# Autodesk Inventor assembly: Main Assembly
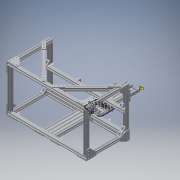
[picture p0: Inventor's stored thumbnail of the model, 180x180]
Saved by Autodesk Inventor 2016 (Build 200138000, 138)
## iProperties
Created: 2016-03-20
Part Number: Main Assembly
Document SubType Name: Assembly
Designer: Solomon
Author: Solomon
## Documents named in this file (13)
- C:\Users\Solomon\Documents\Inventor\SLA MK I\Main Assembly.iam
- C:\Users\Solomon\Documents\Inventor\SLA MK I\V Slot Part Files\Extrusions\vslot 20 x 80 - 500 mm.ipt
- C:\Users\Solomon\Documents\Inventor\SLA MK I\buildplate.iam
- C:\Users\Solomon\Documents\Inventor\SLA MK I\V Slot Part Files\Extrusions\vslot 20 x 20 v2 - 500mm.ipt
- C:\Users\Solomon\Documents\Inventor\SLA MK I\V Slot Part Files\Extrusions\vslot 20 x 20 v2 - 250mm.ipt
- C:\Users\Solomon\Documents\Inventor\SLA MK I\V Slot Part Files\Brackets and Joining Plates\90 Degree Corner Connector.ipt
- C:\Users\Solomon\Documents\Inventor\SLA MK I\V Slot Part Files\Brackets and Joining Plates\5 Hole 90 Degree Bracket.ipt
- C:\Users\Solomon\Documents\Inventor\SLA MK I\V Slot Part Files\Brackets and Joining Plates\3 Hole Joining Strip Plate.ipt
- C:\Users\Solomon\Documents\Inventor\SLA MK I\V Slot Part Files\Brackets and Joining Plates\5 Hole T Joining Plate.ipt
- C:\Users\Solomon\Documents\Inventor\SLA MK I\100mm m5 threaded.ipt
- C:\Users\Solomon\Documents\Inventor\SLA MK I\vwheel.iam
- C:\Users\Solomon\Documents\Inventor\SLA MK I\Motor pulley holder.ipt
- C:\Users\Solomon\Documents\Inventor\SLA MK I\V Slot Part Files\Brackets and Joining Plates\Universal L Bracket.ipt
## Components (71 placed, 12 different names)
1. vslot 20 x 80 - 500 mm:1 — Angle:1, Mate:1, Flush:1, Angle:2, Flush:2, Flush:8, Mate:6, Angle:40, Angle:41, Angle:42, Angle:43, Flush:71, Mate:53, Mate:54, Flush:72, Flush:73, Flush:74, Mate:56, Flush:76, Mate:83, Flush:89, Mate:85, Flush:90, Mate:86, Angle:59, Mate:87, Flush:93, Angle:62, Mate:89, Flush:94, Mate:91
2. buildplate:1 [sub-assembly] — Angle:1, Mate:1, Flush:1, Angle:52, Mate:58, Flush:77, Angle:56, Angle:57
3. vslot 20 x 20 v2 - 500mm:1 — Angle:2, Flush:2, Mate:3, Flush:3, Flush:4, Flush:5, Flush:6, Mate:4, Flush:8, Mate:6, Flush:15, Mate:9, Mate:10, Flush:16, Flush:17, Flush:32, Mate:22, Flush:34, Flush:36, Flush:37, Angle:58, Flush:91, Flush:92
4. vslot 20 x 20 v2 - 500mm:4 — Mate:5, Flush:7, Flush:9, Flush:12, Mate:49, Flush:63, Flush:66, Flush:67, Flush:69, Mate:84, Angle:61, Mate:88, Angle:63, Mate:90, Flush:95
5. vslot 20 x 20 v2 - 250mm:1 — Mate:3, Flush:3, Flush:4, Flush:9, Angle:6, Mate:7, Flush:10, Flush:11, Angle:15, Flush:31, Mate:21, Angle:16, Flush:33, Angle:28, Mate:52, Mate:69, Flush:82
6. vslot 20 x 20 v2 - 250mm:2 — Flush:5, Flush:6, Mate:4, Mate:5, Flush:7, Angle:3, Angle:4, Angle:5, Flush:13, Mate:8, Flush:14, Mate:12, Angle:17, Angle:18, Flush:35, Mate:23, Flush:38, Mate:24, Angle:37, Mate:50, Flush:65, Angle:38, Mate:51, Mate:71, Flush:83
7. vslot 20 x 20 v2 - 250mm:3 — Angle:6, Mate:7, Flush:10, Flush:11, Angle:7, Angle:8, Mate:11, Flush:29, Flush:30, Angle:25, Angle:27, Flush:47, Flush:64, Flush:70, Mate:64, Flush:80, Mate:66, Flush:81, Mate:67, Mate:75, Mate:77
8. vslot 20 x 20 v2 - 250mm:4 — Angle:4, Flush:12, Flush:13, Mate:8, Flush:18, Flush:19, Mate:13, Angle:13, Angle:19, Flush:68, Angle:53, Mate:60, Angle:54, Mate:62, Mate:73, Mate:79, Mate:82
9. vslot 20 x 20 v2 - 250mm:5 — Angle:5, Flush:14, Flush:15, Mate:9, Flush:24, Mate:19, Flush:25
10. vslot 20 x 20 v2 - 250mm:6 — Angle:3, Mate:10, Flush:16, Flush:17, Flush:45
11. vslot 20 x 20 v2 - 500mm:5 — Angle:7, Flush:24, Mate:19, Flush:25, Flush:26, Flush:27, Mate:20, Flush:28, Flush:40, Flush:43, Flush:46, Mate:32, Mate:34, Mate:36, Mate:39
12. vslot 20 x 20 v2 - 500mm:6 — Angle:8, Mate:11, Flush:18, Mate:12, Mate:15, Mate:16, Flush:22, Flush:23, Mate:68, Mate:70, Mate:72, Mate:74, Flush:86, Mate:78, Flush:87, Mate:80
13. vslot 20 x 20 v2 - 500mm:7 — Flush:19, Mate:13, Angle:9, Mate:17, Mate:18, Flush:20, Flush:21, Mate:59, Flush:78, Angle:55, Mate:61, Mate:63, Flush:79, Mate:65, Flush:85, Mate:76, Mate:81, Flush:88
14. 90 Degree Corner Connector:1 — Angle:12, Mate:18, Angle:13, Flush:20, Angle:14
15. 90 Degree Corner Connector:2 — Angle:11, Angle:12, Mate:17, Flush:21
16. 90 Degree Corner Connector:3 — Angle:9, Angle:10, Angle:11, Mate:15, Flush:22
17. 90 Degree Corner Connector:4 — Angle:10, Mate:16, Angle:14, Flush:23
18. vslot 20 x 20 v2 - 250mm:7 — Flush:26, Flush:27, Mate:20, Angle:20, Angle:21, Flush:39, Mate:25, Angle:22, Angle:23, Flush:41, Mate:26, Angle:29, Angle:30, Mate:30, Flush:49, Flush:50, Mate:31, Mate:46, Mate:48
19. vslot 20 x 20 v2 - 250mm:8 — Flush:28, Flush:29, Flush:30, Angle:24, Flush:44, Mate:27, Angle:26, Mate:28, Flush:48, Mate:29, Flush:51, Flush:52, Mate:33, Mate:42, Mate:44
20. 5 Hole 90 Degree Bracket:1 — Angle:19, Flush:37, Flush:38, Mate:24
21. 5 Hole 90 Degree Bracket:4 — Angle:17, Angle:18, Flush:35, Flush:36, Mate:23
22. 5 Hole 90 Degree Bracket:5 — Angle:16, Flush:33, Mate:22, Flush:34
23. 5 Hole 90 Degree Bracket:6 — Angle:15, Flush:31, Flush:32, Mate:21
24. 5 Hole 90 Degree Bracket:7 — Angle:20, Angle:21, Flush:39, Flush:40, Mate:25, Flush:42
25. 5 Hole 90 Degree Bracket:8 — Angle:22, Angle:23, Flush:41, Flush:42, Mate:26
26. 5 Hole 90 Degree Bracket:9 — Angle:24, Flush:43, Flush:44, Mate:27
27. 5 Hole 90 Degree Bracket:10 — Angle:25, Angle:26, Mate:28, Flush:45, Flush:46
28. 5 Hole 90 Degree Bracket:11 — Angle:27, Angle:28, Flush:47, Flush:48, Mate:29, Angle:31
29. 5 Hole 90 Degree Bracket:13 — Angle:29, Angle:30, Mate:30, Flush:49, Flush:50
30. 3 Hole Joining Strip Plate 3 Hole Joining Strip Plate:1 — Angle:33, Angle:34, Mate:35, Flush:53, Mate:36, Flush:54, Flush:55
31. vslot 20 x 20 v2 - 250mm:9 — Angle:31, Flush:51, Mate:31, Mate:32, Angle:32, Angle:35, Mate:38, Flush:56, Mate:40, Angle:36, Mate:45, Flush:61, Mate:47, Flush:62
32. vslot 20 x 20 v2 - 250mm:10 — Angle:32, Flush:52, Mate:33, Mate:34, Angle:33, Angle:34, Mate:35, Flush:53, Mate:37, Mate:41, Flush:59, Mate:43, Flush:60
33. 3 Hole Joining Strip Plate 3 Hole Joining Strip Plate:5 — Mate:37, Flush:54, Flush:55
34. 3 Hole Joining Strip Plate 3 Hole Joining Strip Plate:6 — Angle:35, Mate:38, Flush:56, Mate:39, Flush:57, Flush:58
35. 3 Hole Joining Strip Plate 3 Hole Joining Strip Plate:7 — Mate:40, Flush:57, Flush:58
36. 3 Hole Joining Strip Plate 3 Hole Joining Strip Plate:8 — Mate:41, Flush:59, Mate:42
37. 3 Hole Joining Strip Plate 3 Hole Joining Strip Plate:9 — Mate:43, Mate:44, Flush:60
38. 3 Hole Joining Strip Plate 3 Hole Joining Strip Plate:10 — Angle:36, Mate:45, Flush:61, Mate:46
39. 3 Hole Joining Strip Plate 3 Hole Joining Strip Plate:11 — Mate:47, Flush:62, Mate:48
40. 5 Hole 90 Degree Bracket:14 — Mate:49, Flush:63, Flush:64
41. 5 Hole 90 Degree Bracket:15 — Angle:37, Mate:50, Flush:65, Flush:66, Angle:39
42. 5 Hole T Joining Plate:1 — Angle:38, Angle:39, Mate:51, Flush:67, Flush:68
43. 5 Hole T Joining Plate:2 — Mate:52, Flush:69, Flush:70
44. 3 Hole Joining Strip Plate 3 Hole Joining Strip Plate:12 — Angle:40, Angle:41, Mate:54, Flush:72, Flush:73, Mate:57, Flush:75
45. 3 Hole Joining Strip Plate 3 Hole Joining Strip Plate:13 — Angle:42, Angle:43, Flush:71, Mate:53, Flush:74, Angle:44, Mate:55, Insert:1, Angle:49, Angle:50, Angle:51
46. 3 Hole Joining Strip Plate 3 Hole Joining Strip Plate:14 — Angle:44, Angle:45, Mate:55, Flush:76, Angle:46, Angle:47, Angle:48, Insert:2, Insert:3, Mate:85
47. 3 Hole Joining Strip Plate 3 Hole Joining Strip Plate:15 — Angle:45, Mate:56, Mate:57, Flush:75
48. 100mm m5 threaded:1 — Angle:48, Insert:3, Insert:5
49. 100mm m5 threaded:2 — Angle:47, Insert:2, Insert:6
50. 100mm m5 threaded:3 — Angle:46, Insert:1, Insert:4
51. vwheel:1 [sub-assembly] — Angle:50, Insert:5
52. vwheel:2 [sub-assembly] — Angle:49, Insert:6
53. vwheel:3 [sub-assembly] — Angle:51, Insert:4
54. 5 Hole T Joining Plate:3 — Angle:52, Mate:58, Flush:77
55. 90 Degree Corner Connector:5 — Angle:53, Mate:59, Mate:60, Flush:78
56. 90 Degree Corner Connector:6 — Angle:54, Angle:55, Mate:61, Mate:62
57. 90 Degree Corner Connector:7 — Mate:63, Mate:64, Flush:79
58. 90 Degree Corner Connector:8 — Flush:80, Mate:65, Mate:66
59. 90 Degree Corner Connector:9 — Flush:81, Mate:67, Mate:68
60. 90 Degree Corner Connector:10 — Mate:69, Flush:82, Mate:70
61. 90 Degree Corner Connector:11 — Mate:71, Flush:83, Mate:72, Flush:84
62. 90 Degree Corner Connector:12 — Flush:84, Mate:73, Mate:74
63. 90 Degree Corner Connector:13 — Mate:75, Flush:85, Mate:76
64. 90 Degree Corner Connector:14 — Mate:77, Flush:86, Mate:78
65. 90 Degree Corner Connector:15 — Flush:87, Mate:79, Mate:80
66. 90 Degree Corner Connector:16 — Mate:81, Mate:82, Flush:88
67. Motor pulley holder:1 — Angle:56, Mate:83, Angle:57, Flush:89, Mate:84
68. 5 Hole 90 Degree Bracket:16 — Angle:59, Angle:60, Flush:92, Mate:87, Flush:93
69. 5 Hole 90 Degree Bracket:17 — Angle:58, Flush:90, Mate:86, Flush:91, Angle:60
70. Universal L Bracket:1 — Angle:61, Angle:62, Mate:88, Mate:89, Flush:94
71. 90 Degree Corner Connector:17 — Angle:63, Mate:90, Flush:95, Mate:91
## Relationships (253: Flush 95, Mate 89, Angle 63, Insert 6)
- Angle:1 (0 deg): vslot 20 x 80 - 500 mm:1 ↔ buildplate:1
- Mate:1 (1.5 mm): vslot 20 x 80 - 500 mm:1 ↔ buildplate:1
- Flush:1 (-23.5 mm): vslot 20 x 80 - 500 mm:1 ↔ buildplate:1
- Angle:2 (0 deg): vslot 20 x 80 - 500 mm:1 ↔ vslot 20 x 20 v2 - 500mm:1
- Flush:2 (-210 mm): vslot 20 x 80 - 500 mm:1 ↔ vslot 20 x 20 v2 - 500mm:1
- Mate:3: vslot 20 x 20 v2 - 500mm:1 ↔ vslot 20 x 20 v2 - 250mm:1
- Flush:3: vslot 20 x 20 v2 - 500mm:1 ↔ vslot 20 x 20 v2 - 250mm:1
- Flush:4: vslot 20 x 20 v2 - 500mm:1 ↔ vslot 20 x 20 v2 - 250mm:1
- Flush:5: vslot 20 x 20 v2 - 500mm:1 ↔ vslot 20 x 20 v2 - 250mm:2
- Flush:6: vslot 20 x 20 v2 - 500mm:1 ↔ vslot 20 x 20 v2 - 250mm:2
- Mate:4: vslot 20 x 20 v2 - 500mm:1 ↔ vslot 20 x 20 v2 - 250mm:2
- Mate:5: vslot 20 x 20 v2 - 500mm:4 ↔ vslot 20 x 20 v2 - 250mm:2
- Flush:7: vslot 20 x 20 v2 - 500mm:4 ↔ vslot 20 x 20 v2 - 250mm:2
- Flush:8: vslot 20 x 80 - 500 mm:1 ↔ vslot 20 x 20 v2 - 500mm:1
- Mate:6: vslot 20 x 80 - 500 mm:1 ↔ vslot 20 x 20 v2 - 500mm:1
- Flush:9: vslot 20 x 20 v2 - 500mm:4 ↔ vslot 20 x 20 v2 - 250mm:1
- Angle:3 (0 deg): vslot 20 x 20 v2 - 250mm:2 ↔ vslot 20 x 20 v2 - 250mm:6
- Angle:4 (0 deg): vslot 20 x 20 v2 - 250mm:2 ↔ vslot 20 x 20 v2 - 250mm:4
- Angle:5 (0 deg): vslot 20 x 20 v2 - 250mm:2 ↔ vslot 20 x 20 v2 - 250mm:5
- Angle:6 (0 deg): vslot 20 x 20 v2 - 250mm:1 ↔ vslot 20 x 20 v2 - 250mm:3
- Mate:7: vslot 20 x 20 v2 - 250mm:1 ↔ vslot 20 x 20 v2 - 250mm:3
- Flush:10: vslot 20 x 20 v2 - 250mm:1 ↔ vslot 20 x 20 v2 - 250mm:3
- Flush:11: vslot 20 x 20 v2 - 250mm:1 ↔ vslot 20 x 20 v2 - 250mm:3
- Flush:12: vslot 20 x 20 v2 - 500mm:4 ↔ vslot 20 x 20 v2 - 250mm:4
- Flush:13: vslot 20 x 20 v2 - 250mm:2 ↔ vslot 20 x 20 v2 - 250mm:4
- Mate:8: vslot 20 x 20 v2 - 250mm:2 ↔ vslot 20 x 20 v2 - 250mm:4
- Flush:14: vslot 20 x 20 v2 - 250mm:2 ↔ vslot 20 x 20 v2 - 250mm:5
- Flush:15: vslot 20 x 20 v2 - 500mm:1 ↔ vslot 20 x 20 v2 - 250mm:5
- Mate:9: vslot 20 x 20 v2 - 500mm:1 ↔ vslot 20 x 20 v2 - 250mm:5
- Mate:10: vslot 20 x 20 v2 - 500mm:1 ↔ vslot 20 x 20 v2 - 250mm:6
- Flush:16: vslot 20 x 20 v2 - 500mm:1 ↔ vslot 20 x 20 v2 - 250mm:6
- Flush:17: vslot 20 x 20 v2 - 500mm:1 ↔ vslot 20 x 20 v2 - 250mm:6
- Angle:7 (0 deg): vslot 20 x 20 v2 - 250mm:3 ↔ vslot 20 x 20 v2 - 500mm:5
- Angle:8 (0 deg): vslot 20 x 20 v2 - 250mm:3 ↔ vslot 20 x 20 v2 - 500mm:6
- Mate:11: vslot 20 x 20 v2 - 250mm:3 ↔ vslot 20 x 20 v2 - 500mm:6
- Flush:18: vslot 20 x 20 v2 - 250mm:4 ↔ vslot 20 x 20 v2 - 500mm:6
- Mate:12: vslot 20 x 20 v2 - 250mm:2 ↔ vslot 20 x 20 v2 - 500mm:6
- Flush:19: vslot 20 x 20 v2 - 250mm:4 ↔ vslot 20 x 20 v2 - 500mm:7
- Mate:13: vslot 20 x 20 v2 - 250mm:4 ↔ vslot 20 x 20 v2 - 500mm:7
- Angle:9 (180 deg): vslot 20 x 20 v2 - 500mm:7 ↔ 90 Degree Corner Connector:3
- Angle:10 (0 deg): 90 Degree Corner Connector:3 ↔ 90 Degree Corner Connector:4
- Angle:11 (0 deg): 90 Degree Corner Connector:2 ↔ 90 Degree Corner Connector:3
- Angle:12 (0 deg): 90 Degree Corner Connector:1 ↔ 90 Degree Corner Connector:2
- Mate:15: vslot 20 x 20 v2 - 500mm:6 ↔ 90 Degree Corner Connector:3
- Mate:16: vslot 20 x 20 v2 - 500mm:6 ↔ 90 Degree Corner Connector:4
- Mate:17: vslot 20 x 20 v2 - 500mm:7 ↔ 90 Degree Corner Connector:2
- Mate:18: vslot 20 x 20 v2 - 500mm:7 ↔ 90 Degree Corner Connector:1
- Angle:13 (0 deg): vslot 20 x 20 v2 - 250mm:4 ↔ 90 Degree Corner Connector:1
- Flush:20: vslot 20 x 20 v2 - 500mm:7 ↔ 90 Degree Corner Connector:1
- Flush:21: vslot 20 x 20 v2 - 500mm:7 ↔ 90 Degree Corner Connector:2
- Flush:22: vslot 20 x 20 v2 - 500mm:6 ↔ 90 Degree Corner Connector:3
- Angle:14 (0 deg): 90 Degree Corner Connector:1 ↔ 90 Degree Corner Connector:4
- Flush:23: vslot 20 x 20 v2 - 500mm:6 ↔ 90 Degree Corner Connector:4
- Flush:24: vslot 20 x 20 v2 - 250mm:5 ↔ vslot 20 x 20 v2 - 500mm:5
- Mate:19: vslot 20 x 20 v2 - 250mm:5 ↔ vslot 20 x 20 v2 - 500mm:5
- Flush:25: vslot 20 x 20 v2 - 250mm:5 ↔ vslot 20 x 20 v2 - 500mm:5
- Flush:26: vslot 20 x 20 v2 - 500mm:5 ↔ vslot 20 x 20 v2 - 250mm:7
- Flush:27: vslot 20 x 20 v2 - 500mm:5 ↔ vslot 20 x 20 v2 - 250mm:7
- Mate:20: vslot 20 x 20 v2 - 500mm:5 ↔ vslot 20 x 20 v2 - 250mm:7
- Flush:28: vslot 20 x 20 v2 - 500mm:5 ↔ vslot 20 x 20 v2 - 250mm:8
- Flush:29: vslot 20 x 20 v2 - 250mm:3 ↔ vslot 20 x 20 v2 - 250mm:8
- Flush:30: vslot 20 x 20 v2 - 250mm:3 ↔ vslot 20 x 20 v2 - 250mm:8
- Angle:15 (0 deg): vslot 20 x 20 v2 - 250mm:1 ↔ 5 Hole 90 Degree Bracket:6
- Flush:31: vslot 20 x 20 v2 - 250mm:1 ↔ 5 Hole 90 Degree Bracket:6
- Flush:32: vslot 20 x 20 v2 - 500mm:1 ↔ 5 Hole 90 Degree Bracket:6
- Mate:21: vslot 20 x 20 v2 - 250mm:1 ↔ 5 Hole 90 Degree Bracket:6
- Angle:16 (0 deg): vslot 20 x 20 v2 - 250mm:1 ↔ 5 Hole 90 Degree Bracket:5
- Flush:33: vslot 20 x 20 v2 - 250mm:1 ↔ 5 Hole 90 Degree Bracket:5
- Mate:22: vslot 20 x 20 v2 - 500mm:1 ↔ 5 Hole 90 Degree Bracket:5
- Flush:34: vslot 20 x 20 v2 - 500mm:1 ↔ 5 Hole 90 Degree Bracket:5
- Angle:17 (0 deg): vslot 20 x 20 v2 - 250mm:2 ↔ 5 Hole 90 Degree Bracket:4
- Angle:18 (0 deg): vslot 20 x 20 v2 - 250mm:2 ↔ 5 Hole 90 Degree Bracket:4
- Flush:35: vslot 20 x 20 v2 - 250mm:2 ↔ 5 Hole 90 Degree Bracket:4
- Flush:36: vslot 20 x 20 v2 - 500mm:1 ↔ 5 Hole 90 Degree Bracket:4
- Mate:23: vslot 20 x 20 v2 - 250mm:2 ↔ 5 Hole 90 Degree Bracket:4
- Angle:19 (0 deg): vslot 20 x 20 v2 - 250mm:4 ↔ 5 Hole 90 Degree Bracket:1
- Flush:37: vslot 20 x 20 v2 - 500mm:1 ↔ 5 Hole 90 Degree Bracket:1
- Flush:38: vslot 20 x 20 v2 - 250mm:2 ↔ 5 Hole 90 Degree Bracket:1
- Mate:24: vslot 20 x 20 v2 - 250mm:2 ↔ 5 Hole 90 Degree Bracket:1
- Angle:20 (0 deg): vslot 20 x 20 v2 - 250mm:7 ↔ 5 Hole 90 Degree Bracket:7
- Angle:21 (0 deg): vslot 20 x 20 v2 - 250mm:7 ↔ 5 Hole 90 Degree Bracket:7
- Flush:39: vslot 20 x 20 v2 - 250mm:7 ↔ 5 Hole 90 Degree Bracket:7
- Flush:40: vslot 20 x 20 v2 - 500mm:5 ↔ 5 Hole 90 Degree Bracket:7
- Mate:25: vslot 20 x 20 v2 - 250mm:7 ↔ 5 Hole 90 Degree Bracket:7
- Angle:22 (0 deg): vslot 20 x 20 v2 - 250mm:7 ↔ 5 Hole 90 Degree Bracket:8
- Angle:23 (0 deg): vslot 20 x 20 v2 - 250mm:7 ↔ 5 Hole 90 Degree Bracket:8
- Flush:41: vslot 20 x 20 v2 - 250mm:7 ↔ 5 Hole 90 Degree Bracket:8
- Flush:42: 5 Hole 90 Degree Bracket:7 ↔ 5 Hole 90 Degree Bracket:8
- Mate:26: vslot 20 x 20 v2 - 250mm:7 ↔ 5 Hole 90 Degree Bracket:8
- Angle:24 (0 deg): vslot 20 x 20 v2 - 250mm:8 ↔ 5 Hole 90 Degree Bracket:9
- Flush:43: vslot 20 x 20 v2 - 500mm:5 ↔ 5 Hole 90 Degree Bracket:9
- Flush:44: vslot 20 x 20 v2 - 250mm:8 ↔ 5 Hole 90 Degree Bracket:9
- Mate:27: vslot 20 x 20 v2 - 250mm:8 ↔ 5 Hole 90 Degree Bracket:9
- Angle:25 (0 deg): vslot 20 x 20 v2 - 250mm:3 ↔ 5 Hole 90 Degree Bracket:10
- Angle:26 (180 deg): vslot 20 x 20 v2 - 250mm:8 ↔ 5 Hole 90 Degree Bracket:10
- Mate:28: vslot 20 x 20 v2 - 250mm:8 ↔ 5 Hole 90 Degree Bracket:10
- Flush:45: vslot 20 x 20 v2 - 250mm:6 ↔ 5 Hole 90 Degree Bracket:10
- Flush:46: vslot 20 x 20 v2 - 500mm:5 ↔ 5 Hole 90 Degree Bracket:10
- Angle:27 (0 deg): vslot 20 x 20 v2 - 250mm:3 ↔ 5 Hole 90 Degree Bracket:11
- Angle:28 (0 deg): vslot 20 x 20 v2 - 250mm:1 ↔ 5 Hole 90 Degree Bracket:11
- Flush:47: vslot 20 x 20 v2 - 250mm:3 ↔ 5 Hole 90 Degree Bracket:11
- Flush:48: vslot 20 x 20 v2 - 250mm:8 ↔ 5 Hole 90 Degree Bracket:11
- Mate:29: vslot 20 x 20 v2 - 250mm:8 ↔ 5 Hole 90 Degree Bracket:11
- Angle:29 (0 deg): vslot 20 x 20 v2 - 250mm:7 ↔ 5 Hole 90 Degree Bracket:13
- Angle:30 (180 deg): vslot 20 x 20 v2 - 250mm:7 ↔ 5 Hole 90 Degree Bracket:13
- Mate:30: vslot 20 x 20 v2 - 250mm:7 ↔ 5 Hole 90 Degree Bracket:13
- Flush:49: vslot 20 x 20 v2 - 250mm:7 ↔ 5 Hole 90 Degree Bracket:13
- Flush:50: vslot 20 x 20 v2 - 250mm:7 ↔ 5 Hole 90 Degree Bracket:13
- Angle:31 (45 deg): 5 Hole 90 Degree Bracket:11 ↔ vslot 20 x 20 v2 - 250mm:9
- Flush:51: vslot 20 x 20 v2 - 250mm:8 ↔ vslot 20 x 20 v2 - 250mm:9
- Mate:31: vslot 20 x 20 v2 - 250mm:7 ↔ vslot 20 x 20 v2 - 250mm:9
- Mate:32: vslot 20 x 20 v2 - 500mm:5 ↔ vslot 20 x 20 v2 - 250mm:9
- Angle:32 (90 deg): vslot 20 x 20 v2 - 250mm:9 ↔ vslot 20 x 20 v2 - 250mm:10
- Flush:52: vslot 20 x 20 v2 - 250mm:8 ↔ vslot 20 x 20 v2 - 250mm:10
- Mate:33: vslot 20 x 20 v2 - 250mm:8 ↔ vslot 20 x 20 v2 - 250mm:10
- Mate:34: vslot 20 x 20 v2 - 500mm:5 ↔ vslot 20 x 20 v2 - 250mm:10
- Angle:33 (0 deg): 3 Hole Joining Strip Plate 3 Hole Joining Strip Plate:1 ↔ vslot 20 x 20 v2 - 250mm:10
- Angle:34 (0 deg): 3 Hole Joining Strip Plate 3 Hole Joining Strip Plate:1 ↔ vslot 20 x 20 v2 - 250mm:10
- Mate:35: 3 Hole Joining Strip Plate 3 Hole Joining Strip Plate:1 ↔ vslot 20 x 20 v2 - 250mm:10
- Flush:53: 3 Hole Joining Strip Plate 3 Hole Joining Strip Plate:1 ↔ vslot 20 x 20 v2 - 250mm:10
- Mate:36: vslot 20 x 20 v2 - 500mm:5 ↔ 3 Hole Joining Strip Plate 3 Hole Joining Strip Plate:1
- Mate:37: vslot 20 x 20 v2 - 250mm:10 ↔ 3 Hole Joining Strip Plate 3 Hole Joining Strip Plate:5
- Flush:54: 3 Hole Joining Strip Plate 3 Hole Joining Strip Plate:1 ↔ 3 Hole Joining Strip Plate 3 Hole Joining Strip Plate:5
- Flush:55: 3 Hole Joining Strip Plate 3 Hole Joining Strip Plate:1 ↔ 3 Hole Joining Strip Plate 3 Hole Joining Strip Plate:5
- Angle:35 (0 deg): vslot 20 x 20 v2 - 250mm:9 ↔ 3 Hole Joining Strip Plate 3 Hole Joining Strip Plate:6
- Mate:38: vslot 20 x 20 v2 - 250mm:9 ↔ 3 Hole Joining Strip Plate 3 Hole Joining Strip Plate:6
- Flush:56: vslot 20 x 20 v2 - 250mm:9 ↔ 3 Hole Joining Strip Plate 3 Hole Joining Strip Plate:6
- Mate:39: vslot 20 x 20 v2 - 500mm:5 ↔ 3 Hole Joining Strip Plate 3 Hole Joining Strip Plate:6
- Mate:40: vslot 20 x 20 v2 - 250mm:9 ↔ 3 Hole Joining Strip Plate 3 Hole Joining Strip Plate:7
- Flush:57: 3 Hole Joining Strip Plate 3 Hole Joining Strip Plate:6 ↔ 3 Hole Joining Strip Plate 3 Hole Joining Strip Plate:7
- Flush:58: 3 Hole Joining Strip Plate 3 Hole Joining Strip Plate:6 ↔ 3 Hole Joining Strip Plate 3 Hole Joining Strip Plate:7
- Mate:41: vslot 20 x 20 v2 - 250mm:10 ↔ 3 Hole Joining Strip Plate 3 Hole Joining Strip Plate:8
- Flush:59: vslot 20 x 20 v2 - 250mm:10 ↔ 3 Hole Joining Strip Plate 3 Hole Joining Strip Plate:8
- Mate:42: vslot 20 x 20 v2 - 250mm:8 ↔ 3 Hole Joining Strip Plate 3 Hole Joining Strip Plate:8
- Mate:43: vslot 20 x 20 v2 - 250mm:10 ↔ 3 Hole Joining Strip Plate 3 Hole Joining Strip Plate:9
- Mate:44: vslot 20 x 20 v2 - 250mm:8 ↔ 3 Hole Joining Strip Plate 3 Hole Joining Strip Plate:9
- Flush:60: vslot 20 x 20 v2 - 250mm:10 ↔ 3 Hole Joining Strip Plate 3 Hole Joining Strip Plate:9
- Angle:36 (0 deg): vslot 20 x 20 v2 - 250mm:9 ↔ 3 Hole Joining Strip Plate 3 Hole Joining Strip Plate:10
- Mate:45: vslot 20 x 20 v2 - 250mm:9 ↔ 3 Hole Joining Strip Plate 3 Hole Joining Strip Plate:10
- Flush:61: vslot 20 x 20 v2 - 250mm:9 ↔ 3 Hole Joining Strip Plate 3 Hole Joining Strip Plate:10
- Mate:46: vslot 20 x 20 v2 - 250mm:7 ↔ 3 Hole Joining Strip Plate 3 Hole Joining Strip Plate:10
- Mate:47: vslot 20 x 20 v2 - 250mm:9 ↔ 3 Hole Joining Strip Plate 3 Hole Joining Strip Plate:11
- Flush:62: vslot 20 x 20 v2 - 250mm:9 ↔ 3 Hole Joining Strip Plate 3 Hole Joining Strip Plate:11
- Mate:48: vslot 20 x 20 v2 - 250mm:7 ↔ 3 Hole Joining Strip Plate 3 Hole Joining Strip Plate:11
- Mate:49: vslot 20 x 20 v2 - 500mm:4 ↔ 5 Hole 90 Degree Bracket:14
- Flush:63: vslot 20 x 20 v2 - 500mm:4 ↔ 5 Hole 90 Degree Bracket:14
- Flush:64: vslot 20 x 20 v2 - 250mm:3 ↔ 5 Hole 90 Degree Bracket:14
- Angle:37 (0 deg): vslot 20 x 20 v2 - 250mm:2 ↔ 5 Hole 90 Degree Bracket:15
- Mate:50: vslot 20 x 20 v2 - 250mm:2 ↔ 5 Hole 90 Degree Bracket:15
- Flush:65: vslot 20 x 20 v2 - 250mm:2 ↔ 5 Hole 90 Degree Bracket:15
- Flush:66: vslot 20 x 20 v2 - 500mm:4 ↔ 5 Hole 90 Degree Bracket:15
- Angle:38 (0 deg): vslot 20 x 20 v2 - 250mm:2 ↔ 5 Hole T Joining Plate:1
- Angle:39 (0 deg): 5 Hole 90 Degree Bracket:15 ↔ 5 Hole T Joining Plate:1
- Mate:51: vslot 20 x 20 v2 - 250mm:2 ↔ 5 Hole T Joining Plate:1
- Flush:67: vslot 20 x 20 v2 - 500mm:4 ↔ 5 Hole T Joining Plate:1
- Flush:68: vslot 20 x 20 v2 - 250mm:4 ↔ 5 Hole T Joining Plate:1
- Mate:52: vslot 20 x 20 v2 - 250mm:1 ↔ 5 Hole T Joining Plate:2
- Flush:69: vslot 20 x 20 v2 - 500mm:4 ↔ 5 Hole T Joining Plate:2
- Flush:70: vslot 20 x 20 v2 - 250mm:3 ↔ 5 Hole T Joining Plate:2
- Angle:40 (0 deg): vslot 20 x 80 - 500 mm:1 ↔ 3 Hole Joining Strip Plate 3 Hole Joining Strip Plate:12
- Angle:41 (0 deg): vslot 20 x 80 - 500 mm:1 ↔ 3 Hole Joining Strip Plate 3 Hole Joining Strip Plate:12
- Angle:42 (0 deg): vslot 20 x 80 - 500 mm:1 ↔ 3 Hole Joining Strip Plate 3 Hole Joining Strip Plate:13
- Angle:43 (0 deg): vslot 20 x 80 - 500 mm:1 ↔ 3 Hole Joining Strip Plate 3 Hole Joining Strip Plate:13
- Flush:71: vslot 20 x 80 - 500 mm:1 ↔ 3 Hole Joining Strip Plate 3 Hole Joining Strip Plate:13
- Mate:53: vslot 20 x 80 - 500 mm:1 ↔ 3 Hole Joining Strip Plate 3 Hole Joining Strip Plate:13
- Mate:54: vslot 20 x 80 - 500 mm:1 ↔ 3 Hole Joining Strip Plate 3 Hole Joining Strip Plate:12
- Flush:72: vslot 20 x 80 - 500 mm:1 ↔ 3 Hole Joining Strip Plate 3 Hole Joining Strip Plate:12
- Flush:73 (-25 mm): vslot 20 x 80 - 500 mm:1 ↔ 3 Hole Joining Strip Plate 3 Hole Joining Strip Plate:12
- Flush:74 (-25 mm): vslot 20 x 80 - 500 mm:1 ↔ 3 Hole Joining Strip Plate 3 Hole Joining Strip Plate:13
- Angle:44 (0 deg): 3 Hole Joining Strip Plate 3 Hole Joining Strip Plate:13 ↔ 3 Hole Joining Strip Plate 3 Hole Joining Strip Plate:14
- Angle:45 (0 deg): 3 Hole Joining Strip Plate 3 Hole Joining Strip Plate:14 ↔ 3 Hole Joining Strip Plate 3 Hole Joining Strip Plate:15
- Mate:55: 3 Hole Joining Strip Plate 3 Hole Joining Strip Plate:13 ↔ 3 Hole Joining Strip Plate 3 Hole Joining Strip Plate:14
- Mate:56: vslot 20 x 80 - 500 mm:1 ↔ 3 Hole Joining Strip Plate 3 Hole Joining Strip Plate:15
- Mate:57: 3 Hole Joining Strip Plate 3 Hole Joining Strip Plate:12 ↔ 3 Hole Joining Strip Plate 3 Hole Joining Strip Plate:15
- Flush:75 (20 mm): 3 Hole Joining Strip Plate 3 Hole Joining Strip Plate:12 ↔ 3 Hole Joining Strip Plate 3 Hole Joining Strip Plate:15
- Flush:76 (-20 mm): vslot 20 x 80 - 500 mm:1 ↔ 3 Hole Joining Strip Plate 3 Hole Joining Strip Plate:14
- Angle:46 (0 deg): 3 Hole Joining Strip Plate 3 Hole Joining Strip Plate:14 ↔ 100mm m5 threaded:3
- Angle:47 (0 deg): 3 Hole Joining Strip Plate 3 Hole Joining Strip Plate:14 ↔ 100mm m5 threaded:2
- Angle:48 (0 deg): 3 Hole Joining Strip Plate 3 Hole Joining Strip Plate:14 ↔ 100mm m5 threaded:1
- Insert:1 (-5 mm): 3 Hole Joining Strip Plate 3 Hole Joining Strip Plate:13 ↔ 100mm m5 threaded:3
- Insert:2 (-5 mm): 3 Hole Joining Strip Plate 3 Hole Joining Strip Plate:14 ↔ 100mm m5 threaded:2
- Insert:3 (-5 mm): 3 Hole Joining Strip Plate 3 Hole Joining Strip Plate:14 ↔ 100mm m5 threaded:1
- Angle:49 (0 deg): 3 Hole Joining Strip Plate 3 Hole Joining Strip Plate:13 ↔ vwheel:2
- Angle:50 (0 deg): 3 Hole Joining Strip Plate 3 Hole Joining Strip Plate:13 ↔ vwheel:1
- Angle:51 (0 deg): 3 Hole Joining Strip Plate 3 Hole Joining Strip Plate:13 ↔ vwheel:3
- Insert:4 (-50 mm): 100mm m5 threaded:3 ↔ vwheel:3
- Insert:5 (-50 mm): 100mm m5 threaded:1 ↔ vwheel:1
- Insert:6 (-50 mm): 100mm m5 threaded:2 ↔ vwheel:2
- Angle:52 (0 deg): buildplate:1 ↔ 5 Hole T Joining Plate:3
- Mate:58: buildplate:1 ↔ 5 Hole T Joining Plate:3
- Flush:77 (33.5 mm): buildplate:1 ↔ 5 Hole T Joining Plate:3
- Angle:53 (180 deg): vslot 20 x 20 v2 - 250mm:4 ↔ 90 Degree Corner Connector:5
- Mate:59: vslot 20 x 20 v2 - 500mm:7 ↔ 90 Degree Corner Connector:5
- Mate:60: vslot 20 x 20 v2 - 250mm:4 ↔ 90 Degree Corner Connector:5
- Flush:78: vslot 20 x 20 v2 - 500mm:7 ↔ 90 Degree Corner Connector:5
- Angle:54 (90 deg): vslot 20 x 20 v2 - 250mm:4 ↔ 90 Degree Corner Connector:6
- Angle:55 (0 deg): vslot 20 x 20 v2 - 500mm:7 ↔ 90 Degree Corner Connector:6
- Mate:61: vslot 20 x 20 v2 - 500mm:7 ↔ 90 Degree Corner Connector:6
- Mate:62: vslot 20 x 20 v2 - 250mm:4 ↔ 90 Degree Corner Connector:6
- Mate:63: vslot 20 x 20 v2 - 500mm:7 ↔ 90 Degree Corner Connector:7
- Mate:64: vslot 20 x 20 v2 - 250mm:3 ↔ 90 Degree Corner Connector:7
- Flush:79: vslot 20 x 20 v2 - 500mm:7 ↔ 90 Degree Corner Connector:7
- Flush:80: vslot 20 x 20 v2 - 250mm:3 ↔ 90 Degree Corner Connector:8
- Mate:65: vslot 20 x 20 v2 - 500mm:7 ↔ 90 Degree Corner Connector:8
- Mate:66: vslot 20 x 20 v2 - 250mm:3 ↔ 90 Degree Corner Connector:8
- Flush:81: vslot 20 x 20 v2 - 250mm:3 ↔ 90 Degree Corner Connector:9
- Mate:67: vslot 20 x 20 v2 - 250mm:3 ↔ 90 Degree Corner Connector:9
- Mate:68: vslot 20 x 20 v2 - 500mm:6 ↔ 90 Degree Corner Connector:9
- Mate:69: vslot 20 x 20 v2 - 250mm:1 ↔ 90 Degree Corner Connector:10
- Flush:82: vslot 20 x 20 v2 - 250mm:1 ↔ 90 Degree Corner Connector:10
- Mate:70: vslot 20 x 20 v2 - 500mm:6 ↔ 90 Degree Corner Connector:10
- Mate:71: vslot 20 x 20 v2 - 250mm:2 ↔ 90 Degree Corner Connector:11
- Flush:83: vslot 20 x 20 v2 - 250mm:2 ↔ 90 Degree Corner Connector:11
- Mate:72: vslot 20 x 20 v2 - 500mm:6 ↔ 90 Degree Corner Connector:11
- Flush:84: 90 Degree Corner Connector:11 ↔ 90 Degree Corner Connector:12
- Mate:73: vslot 20 x 20 v2 - 250mm:4 ↔ 90 Degree Corner Connector:12
- Mate:74: vslot 20 x 20 v2 - 500mm:6 ↔ 90 Degree Corner Connector:12
- Mate:75: vslot 20 x 20 v2 - 250mm:3 ↔ 90 Degree Corner Connector:13
- Flush:85: vslot 20 x 20 v2 - 500mm:7 ↔ 90 Degree Corner Connector:13
- Mate:76: vslot 20 x 20 v2 - 500mm:7 ↔ 90 Degree Corner Connector:13
- Mate:77: vslot 20 x 20 v2 - 250mm:3 ↔ 90 Degree Corner Connector:14
- Flush:86: vslot 20 x 20 v2 - 500mm:6 ↔ 90 Degree Corner Connector:14
- Mate:78: vslot 20 x 20 v2 - 500mm:6 ↔ 90 Degree Corner Connector:14
- Flush:87: vslot 20 x 20 v2 - 500mm:6 ↔ 90 Degree Corner Connector:15
- Mate:79: vslot 20 x 20 v2 - 250mm:4 ↔ 90 Degree Corner Connector:15
- Mate:80: vslot 20 x 20 v2 - 500mm:6 ↔ 90 Degree Corner Connector:15
- Mate:81: vslot 20 x 20 v2 - 500mm:7 ↔ 90 Degree Corner Connector:16
- Mate:82: vslot 20 x 20 v2 - 250mm:4 ↔ 90 Degree Corner Connector:16
- Flush:88: vslot 20 x 20 v2 - 500mm:7 ↔ 90 Degree Corner Connector:16
- Angle:56 (0 deg): buildplate:1 ↔ Motor pulley holder:1
- Mate:83: vslot 20 x 80 - 500 mm:1 ↔ Motor pulley holder:1
- Angle:57 (180 deg): buildplate:1 ↔ Motor pulley holder:1
- Flush:89 (10 mm): vslot 20 x 80 - 500 mm:1 ↔ Motor pulley holder:1
- Mate:84 (25 mm): vslot 20 x 20 v2 - 500mm:4 ↔ Motor pulley holder:1
- Mate:85: vslot 20 x 80 - 500 mm:1 ↔ 3 Hole Joining Strip Plate 3 Hole Joining Strip Plate:14
- Angle:58 (180 deg): vslot 20 x 20 v2 - 500mm:1 ↔ 5 Hole 90 Degree Bracket:17
- Flush:90 (60 mm): vslot 20 x 80 - 500 mm:1 ↔ 5 Hole 90 Degree Bracket:17
- Mate:86: vslot 20 x 80 - 500 mm:1 ↔ 5 Hole 90 Degree Bracket:17
- Flush:91: vslot 20 x 20 v2 - 500mm:1 ↔ 5 Hole 90 Degree Bracket:17
- Angle:59 (180 deg): vslot 20 x 80 - 500 mm:1 ↔ 5 Hole 90 Degree Bracket:16
- Angle:60 (0 deg): 5 Hole 90 Degree Bracket:16 ↔ 5 Hole 90 Degree Bracket:17
- Flush:92: vslot 20 x 20 v2 - 500mm:1 ↔ 5 Hole 90 Degree Bracket:16
- Mate:87: vslot 20 x 80 - 500 mm:1 ↔ 5 Hole 90 Degree Bracket:16
- Flush:93 (-62 mm): vslot 20 x 80 - 500 mm:1 ↔ 5 Hole 90 Degree Bracket:16
- Angle:61 (0 deg): vslot 20 x 20 v2 - 500mm:4 ↔ Universal L Bracket:1
- Angle:62 (0 deg): vslot 20 x 80 - 500 mm:1 ↔ Universal L Bracket:1
- Mate:88: vslot 20 x 20 v2 - 500mm:4 ↔ Universal L Bracket:1
- Mate:89: vslot 20 x 80 - 500 mm:1 ↔ Universal L Bracket:1
- Flush:94: vslot 20 x 80 - 500 mm:1 ↔ Universal L Bracket:1
- Angle:63 (180 deg): vslot 20 x 20 v2 - 500mm:4 ↔ 90 Degree Corner Connector:17
- Mate:90: vslot 20 x 20 v2 - 500mm:4 ↔ 90 Degree Corner Connector:17
- Flush:95: vslot 20 x 20 v2 - 500mm:4 ↔ 90 Degree Corner Connector:17
- Mate:91: vslot 20 x 80 - 500 mm:1 ↔ 90 Degree Corner Connector:17
